# Autodesk Inventor assembly: servo micro asm2
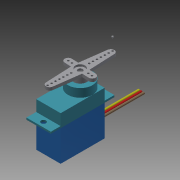
[picture p0: Inventor's stored thumbnail of the model, 180x180]
Saved by Autodesk Inventor 2015 SP2 (Build 190223200, 223)
## iProperties
Created: 2015-05-24
Part Number: servo micro asm2
Document SubType Name: Assembly
Designer: caleb
Author: caleb
## Documents named in this file (3)
- C:\cygwin64\home\caleb\3d\designs\deep-focus-scanning-adapter\servo micro asm2.iam
- C:\cygwin64\home\caleb\3d\designs\deep-focus-scanning-adapter\servo-micro tower pro 9g.ipt
- C:\cygwin64\home\caleb\3d\designs\deep-focus-scanning-adapter\servo micro arm.ipt
## Components (2 placed, 2 different names)
1. servo-micro tower pro 9g:1 — Flush:1, Flush:2, Flush:3, Mate:1, Mate:2
2. servo micro arm:1 — Mate:1, Mate:2
## Relationships (5: Flush 3, Mate 2)
- Flush:1: servo-micro tower pro 9g:1
- Flush:2: servo-micro tower pro 9g:1
- Flush:3: servo-micro tower pro 9g:1
- Mate:1: servo-micro tower pro 9g:1 ↔ servo micro arm:1
- Mate:2: servo-micro tower pro 9g:1 ↔ servo micro arm:1
